# Autodesk Inventor assembly: Y End Stop Assembly
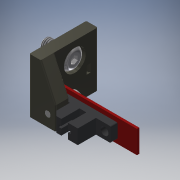
[picture p0: Inventor's stored thumbnail of the model, 180x180]
Saved by Autodesk Inventor 2016 (Build 200138000, 138)
## iProperties
Created: 2017-02-12
Part Number: Y End Stop Assembly
Document SubType Name: Assembly
Designer: Scott
Author: Scott
## Documents named in this file (5)
- E:\Scott Projects\3D Printing\CoreXY\Y End Stop Assembly.iam
- E:\Scott Projects\3D Printing\CoreXY\Y End Stop Bracket.ipt
- E:\Scott Projects\3D Printing\CoreXY\Endstop_Opto_TCST2103.iam
- C:\Users\Scott\Documents\Inventor\Content Center Files\R2016\en-US\ANSI B18.3.4M(1)\ANSI B18.3.4M - M5 x 0.8 x 10(2).ipt
- C:\Users\Scott\Documents\Inventor\Content Center Files\R2016\en-US\AS 1420\AS 1420 - 1973 - M3 x 10.ipt
## Components (4 placed, 4 different names)
1. Y End Stop Bracket:1 — Insert:1, Angle:1, Insert:3
2. Endstop_Opto_TCST2103:1 [sub-assembly] — Insert:1, Angle:1, Insert:2
3. AS 1420 - Metric M3 x 10:1 — Insert:2
4. Broached Hexagon Socket Button Head Cap Screw - Metric M5 x 0.8 x 10:1 — Insert:3
## Relationships (4: Insert 3, Angle 1)
- Insert:1: Y End Stop Bracket:1 ↔ Endstop_Opto_TCST2103:1
- Angle:1 (0 deg): Y End Stop Bracket:1 ↔ Endstop_Opto_TCST2103:1
- Insert:2: Endstop_Opto_TCST2103:1 ↔ AS 1420 - Metric M3 x 10:1
- Insert:3: Y End Stop Bracket:1 ↔ Broached Hexagon Socket Button Head Cap Screw - Metric M5 x 0.8 x 10:1
